# Autodesk Inventor assembly: A.Crankshaft Subassembly
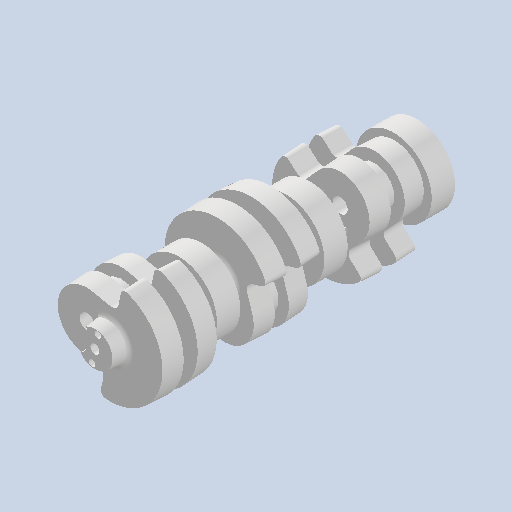
[picture p0: Inventor's stored thumbnail of the model, 512x512]
Saved by Autodesk Inventor 2023 (Build 270158000, 158)
## iProperties
Created: 2023-01-04
Part Number: A.Crankshaft Subassembly
Document SubType Name: Assembly
Designer: tgr41
Author: tgr41
## Documents named in this file (5)
- C:\Users\tommy\Documents\Repositories\Steam-Engine\1.5x1 Inch 3 Cylidner\Old\Cast Engine Block Design V4\A.Crankshaft Subassembly.iam
- C:\Users\tommy\Documents\Repositories\Steam-Engine\1.5x1 Inch 3 Cylidner\Old\Cast Engine Block Design V4\C.Crank on Crankshaft.ipt
- C:\Users\tommy\Documents\Repositories\Steam-Engine\1.5x1 Inch 3 Cylidner\Old\Cast Engine Block Design V4\C.Crank Connect Shaft.ipt
- C:\Users\tommy\Documents\Repositories\Steam-Engine\1.5x1 Inch 3 Cylidner\Old\Cast Engine Block Design V4\C.Crankshaft Main Bearing.ipt
- C:\Users\tommy\Documents\Repositories\Steam-Engine\1.5x1 Inch 3 Cylidner\Old\Cast Engine Block Design V4\C.Connecting Rod Bearing.ipt
## Components (15 placed, 4 different names)
1. C.Crank on Crankshaft:1 — Mate:1, Mate:2, Mate:5, Angle:1, Mate:7, Mate:8
2. C.Crank on Crankshaft:2 — Mate:3, Mate:4, Angle:1, Mate:25, Mate:26, Mate:27
3. C.Crank Connect Shaft:1 — Mate:5, Mate:6, Flush:1, Mate:7, Mate:8
4. C.Crankshaft Main Bearing:2 — Mate:6, Flush:1
5. C.Connecting Rod Bearing:1 — Mate:1, Mate:2, Mate:3, Mate:4
6. C.Crank on Crankshaft:3
7. C.Crank on Crankshaft:4 — Mate:28, Mate:29, Mate:30
8. C.Crank Connect Shaft:2 — Mate:25, Mate:26, Mate:27
9. C.Crankshaft Main Bearing:3
10. C.Connecting Rod Bearing:2
11. C.Crank on Crankshaft:5
12. C.Crank on Crankshaft:6
13. C.Crank Connect Shaft:3 — Mate:28, Mate:29, Mate:30
14. C.Crankshaft Main Bearing:4
15. C.Connecting Rod Bearing:3
## Relationships (36: Mate 30, Flush 3, Angle 3)
- Mate:1: C.Crank on Crankshaft:1 ↔ C.Connecting Rod Bearing:1
- Mate:2: C.Crank on Crankshaft:1 ↔ C.Connecting Rod Bearing:1
- Mate:3: C.Crank on Crankshaft:2 ↔ C.Connecting Rod Bearing:1
- Mate:4: C.Crank on Crankshaft:2 ↔ C.Connecting Rod Bearing:1
- Mate:5: C.Crank on Crankshaft:1 ↔ C.Crank Connect Shaft:1
- Mate:6: C.Crank Connect Shaft:1 ↔ C.Crankshaft Main Bearing:2
- Flush:1: C.Crank Connect Shaft:1 ↔ C.Crankshaft Main Bearing:2
- Angle:1 (0 deg): C.Crank on Crankshaft:1 ↔ C.Crank on Crankshaft:2
- Mate:7: C.Crank on Crankshaft:1 ↔ C.Crank Connect Shaft:1
- Mate:8: C.Crank on Crankshaft:1 ↔ C.Crank Connect Shaft:1
- [Mate]: C.Crank on Crankshaft:3 ↔ C.Connecting Rod Bearing:2
- [Mate]: C.Crank on Crankshaft:3 ↔ C.Connecting Rod Bearing:2
- [Mate]: C.Crank on Crankshaft:4 ↔ C.Connecting Rod Bearing:2
- [Mate]: C.Crank on Crankshaft:4 ↔ C.Connecting Rod Bearing:2
- [Mate]: C.Crank on Crankshaft:3 ↔ C.Crank Connect Shaft:2
- [Mate]: C.Crank Connect Shaft:2 ↔ C.Crankshaft Main Bearing:3
- [Flush]: C.Crank Connect Shaft:2 ↔ C.Crankshaft Main Bearing:3
- [Angle] (0 deg): C.Crank on Crankshaft:3 ↔ C.Crank on Crankshaft:4
- [Mate]: C.Crank on Crankshaft:3 ↔ C.Crank Connect Shaft:2
- [Mate]: C.Crank on Crankshaft:3 ↔ C.Crank Connect Shaft:2
- [Mate]: C.Crank on Crankshaft:5 ↔ C.Connecting Rod Bearing:3
- [Mate]: C.Crank on Crankshaft:5 ↔ C.Connecting Rod Bearing:3
- [Mate]: C.Crank on Crankshaft:6 ↔ C.Connecting Rod Bearing:3
- [Mate]: C.Crank on Crankshaft:6 ↔ C.Connecting Rod Bearing:3
- [Mate]: C.Crank on Crankshaft:5 ↔ C.Crank Connect Shaft:3
- [Mate]: C.Crank Connect Shaft:3 ↔ C.Crankshaft Main Bearing:4
- [Flush]: C.Crank Connect Shaft:3 ↔ C.Crankshaft Main Bearing:4
- [Angle] (0 deg): C.Crank on Crankshaft:5 ↔ C.Crank on Crankshaft:6
- [Mate]: C.Crank on Crankshaft:5 ↔ C.Crank Connect Shaft:3
- [Mate]: C.Crank on Crankshaft:5 ↔ C.Crank Connect Shaft:3
- Mate:25: C.Crank on Crankshaft:2 ↔ C.Crank Connect Shaft:2
- Mate:26: C.Crank on Crankshaft:2 ↔ C.Crank Connect Shaft:2
- Mate:27: C.Crank on Crankshaft:2 ↔ C.Crank Connect Shaft:2
- Mate:28: C.Crank on Crankshaft:4 ↔ C.Crank Connect Shaft:3
- Mate:29: C.Crank on Crankshaft:4 ↔ C.Crank Connect Shaft:3
- Mate:30: C.Crank on Crankshaft:4 ↔ C.Crank Connect Shaft:3
## Named parameters: d10_d0 = 0 mm, d11_d1 = 0 mm, d12_d2 = 0 mm, d13_d3 = 0 mm, d14_d4 = 0 mm, d15_d5 = 0 mm, d16_d6 = 0 mm, d17_d7 = 0 deg, d18_d8 = 0 mm, d19_d9 = 0 mm, d20_d0 = 0 mm, d21_d1 = 0 mm, d22_d2 = 0 mm, d23_d3 = 0 mm, d24_d4 = 0 mm, d25_d5 = 0 mm, d26_d6 = 0 mm, d27_d7 = 0 deg, d28_d8 = 0 mm, d29_d9 = 0 mm
